# Autodesk Inventor assembly: FitAssemby
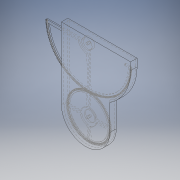
[picture p0: Inventor's stored thumbnail of the model, 180x180]
Saved by Autodesk Inventor 2017 (Build 210142000, 142)
## iProperties
Created: 2016-11-25
Part Number: FitAssemby
Document SubType Name: Assembly
Designer: cody
Author: cody
## Documents named in this file (4)
- C:\Users\cody\Documents\Inventor\mechanism-door-actuator\FitAssemby.iam
- C:\Users\cody\Documents\Inventor\mechanism-door-actuator\arm.ipt
- C:\Users\cody\Documents\Inventor\mechanism-door-actuator\housing.ipt
- C:\Users\cody\Documents\Inventor\mechanism-door-actuator\servo-gear.ipt
## Components (3 placed, 2 different names)
1. arm:1 — Mate:3, Angle:1
2. housing:1 — Mate:1, Angle:1
3. arm:2 — Mate:2
## Relationships (4: Mate 3, Angle 1)
- Mate:1: housing:1
- Mate:2 (-3.175 mm): arm:2
- Mate:3 (-3.175 mm): arm:1
- Angle:1 (0 deg): arm:1 ↔ housing:1
